# Autodesk Inventor assembly: EL2-C-100
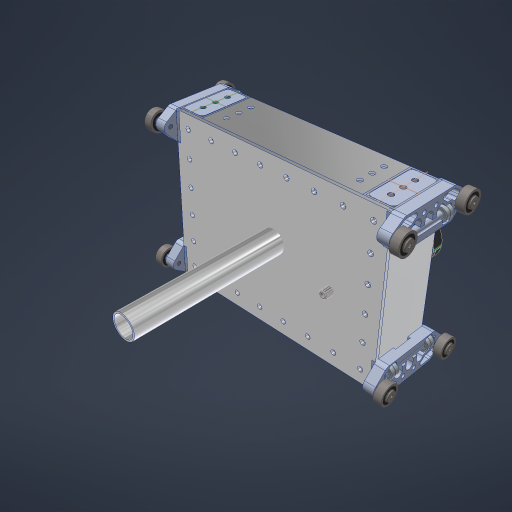
[picture p0: Inventor's stored thumbnail of the model, 512x512]
Saved by Autodesk Inventor 2023.4 (Build 274418000, 418)
## iProperties
Created: 2025-01-11
Part Number: EL2-C-100
Document SubType Name: Assembly
Designer: brand
Author: brand
## Documents named in this file (8)
- C:\Users\brand\OneDrive\Documents\GitHub\robotics 23\2025-ReefScape---CAD\Elevator\EL2\EL2-C-100.iam
- C:\Users\brand\OneDrive\Documents\GitHub\robotics 23\2025-ReefScape---CAD\Elevator\EL2\EL2-C-001.ipt
- C:\Users\brand\OneDrive\Documents\GitHub\robotics 23\2025-ReefScape---CAD\COMMON PARTS\WCP Elevator parts\WCP-0897\WCP-0897.iam
- C:\Users\brand\OneDrive\Documents\GitHub\robotics 23\2025-ReefScape---CAD\Elevator\EL2\EL2-005.ipt
- C:\Users\brand\OneDrive\Documents\GitHub\robotics 23\2025-ReefScape---CAD\Elevator\EL2\EL2-C-003.ipt
- C:\Users\brand\OneDrive\Documents\GitHub\robotics 23\2025-ReefScape---CAD\COMMON PARTS\MOTORS\WCP-0941 x44 Kracken.ipt
- C:\Users\brand\OneDrive\Documents\GitHub\robotics 23\2025-ReefScape---CAD\Elevator\EL2\EL2-C-004.ipt
- C:\Users\brand\OneDrive\Documents\GitHub\robotics 23\2025-ReefScape---CAD\Elevator\EL2\EL2-C-005.ipt
## Components (15 placed, 7 different names)
1. EL2-C-001:1 — Flush:4, Flush:5, Flush:8, Mate:9, Mate:10, Flush:9, Flush:11, Flush:12
2. EL2-C-005:2 — Insert:1, Angle:1, Insert:2, Angle:2, Insert:3, Insert:4, Insert:20, Insert:21, Flush:4, Mate:10
3. EL2-C-005:1 — Insert:8, Angle:3, Insert:9, Insert:10, Angle:4, Insert:22, Insert:23, Flush:5, Mate:8, Flush:7, Mate:9, Mate:11
4. EL2-C-001:4 — Flush:10, Flush:11, Mate:11
5. WCP-0897:1 [sub-assembly] — Insert:9
6. WCP-0897:2 [sub-assembly] — Insert:3, Insert:4
7. EL2-005:1 — Insert:2, Angle:2, Flush:9
8. EL2-005:2 — Insert:8, Angle:3, Flush:8
9. EL2-005:3 — Insert:10, Angle:4, Flush:10
10. EL2-005:4 — Insert:1, Angle:1
11. WCP-0897:3 [sub-assembly] — Insert:22, Insert:23
12. WCP-0897:4 [sub-assembly] — Insert:20, Insert:21
13. EL2-C-003:1 — Mate:8, Flush:7, Flush:12
14. WCP-0941 x44 Kracken:1
15. EL2-C-004:1
## Relationships (27: Insert 11, Flush 8, Angle 4, Mate 4)
- Insert:1: EL2-C-005:2 ↔ EL2-005:4
- Angle:1 (0 deg): EL2-C-005:2 ↔ EL2-005:4
- Insert:2: EL2-C-005:2 ↔ EL2-005:1
- Angle:2 (0 deg): EL2-C-005:2 ↔ EL2-005:1
- Insert:3: EL2-C-005:2 ↔ WCP-0897:2
- Insert:4: EL2-C-005:2 ↔ WCP-0897:2
- Insert:8: EL2-C-005:1 ↔ EL2-005:2
- Angle:3 (0 deg): EL2-C-005:1 ↔ EL2-005:2
- Insert:9: EL2-C-005:1 ↔ WCP-0897:1
- Insert:10: EL2-C-005:1 ↔ EL2-005:3
- Angle:4 (0 deg): EL2-C-005:1 ↔ EL2-005:3
- Insert:20: EL2-C-005:2 ↔ WCP-0897:4
- Insert:21: EL2-C-005:2 ↔ WCP-0897:4
- Insert:22: EL2-C-005:1 ↔ WCP-0897:3
- Insert:23: EL2-C-005:1 ↔ WCP-0897:3
- Flush:4: EL2-C-001:1 ↔ EL2-C-005:2
- Flush:5: EL2-C-001:1 ↔ EL2-C-005:1
- Mate:8: EL2-C-005:1 ↔ EL2-C-003:1
- Flush:7: EL2-C-005:1 ↔ EL2-C-003:1
- Flush:8: EL2-C-001:1 ↔ EL2-005:2
- Mate:9: EL2-C-001:1 ↔ EL2-C-005:1
- Mate:10: EL2-C-001:1 ↔ EL2-C-005:2
- Flush:9: EL2-C-001:1 ↔ EL2-005:1
- Flush:10: EL2-C-001:4 ↔ EL2-005:3
- Flush:11: EL2-C-001:1 ↔ EL2-C-001:4
- Mate:11: EL2-C-005:1 ↔ EL2-C-001:4
- Flush:12: EL2-C-001:1 ↔ EL2-C-003:1
